# Autodesk Inventor assembly: Main Body
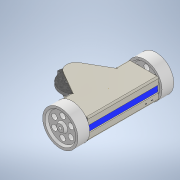
[picture p0: Inventor's stored thumbnail of the model, 180x180]
Saved by Autodesk Inventor 2022 (Build 260153000, 153)
## iProperties
Created: 2022-08-09
Part Number: Main Body
Document SubType Name: Assembly
Designer: Nick
Mass: 1318.27 g
Surface Area: 1845.37 cm^2
Volume: 451.196 cm^3
Density: 2.92172 g/cm^3
Author: Nick
## Documents named in this file (15)
- Y:\Projects\BattleBot\Main Body.iam
- Y:\Projects\BattleBot\Battery.ipt
- Y:\Projects\BattleBot\ESC.ipt
- Y:\Projects\BattleBot\Motor.ipt
- Y:\Projects\BattleBot\RC Reciever.ipt
- Y:\Projects\BattleBot\Base Plate.ipt
- Y:\Projects\BattleBot\Weapon.ipt
- Y:\Projects\BattleBot\Unmodified Motor.ipt
- Y:\Projects\BattleBot\Brushed ESC.ipt
- Y:\Projects\BattleBot\Motor Mount.ipt
- Y:\Projects\BattleBot\Wheel.ipt
- Y:\Projects\BattleBot\6201 Bearing.ipt
- Y:\Projects\BattleBot\Pulley.ipt
- Y:\Projects\BattleBot\6901 Bearing.ipt
- Y:\Projects\BattleBot\pulley flange.ipt
## Components (19 placed, 14 different names)
1. Battery:1 — Mate:65, Mate:66
2. ESC:1 — Mate:66
3. RC Reciever:1 — Mate:53, Mate:62, Mate:64
4. Base Plate:1 — Flush:16, Mate:42, Mate:67, Insert:10
5. Weapon:1 — Insert:3, Mate:70
6. Unmodified Motor:1 — Mate:61
7. Motor:2 — Mate:65, Insert:5, Insert:8
8. Motor:3 — Insert:2, Insert:4
9. Brushed ESC:1
10. Brushed ESC:2 — Mate:55, Mate:56, Mate:63
11. Motor Mount:2 — Insert:2, Flush:16, Mate:42, Mate:53, Mate:55, Mate:56, Mate:62, Mate:63, Mate:64, Mate:67, Insert:8, Mate:68, Mate:69, Flush:17
12. Base Plate:2 — Mate:61, Insert:3, Insert:7, Mate:68, Mate:69, Flush:17
13. Wheel:1 — Insert:5
14. Wheel:2 — Insert:4
15. 6201 Bearing:2 — Insert:7
16. Pulley:1 — Insert:11, Mate:70, Insert:13, Insert:14
17. 6901 Bearing:1 — Insert:10, Insert:14
18. pulley flange:1 — Insert:11
19. pulley flange:2 — Insert:13
## Relationships (26: Mate 14, Insert 10, Flush 2)
- Insert:2: Motor:3 ↔ Motor Mount:2
- Flush:16: Base Plate:1 ↔ Motor Mount:2
- Mate:42: Base Plate:1 ↔ Motor Mount:2
- Mate:53: RC Reciever:1 ↔ Motor Mount:2
- Mate:55: Brushed ESC:2 ↔ Motor Mount:2
- Mate:56: Brushed ESC:2 ↔ Motor Mount:2
- Mate:61: Unmodified Motor:1 ↔ Base Plate:2
- Insert:3 (16.825 mm): Weapon:1 ↔ Base Plate:2
- Mate:62: RC Reciever:1 ↔ Motor Mount:2
- Mate:63 (5 mm): Brushed ESC:2 ↔ Motor Mount:2
- Mate:64: RC Reciever:1 ↔ Motor Mount:2
- Mate:65 (6 mm): Battery:1 ↔ Motor:2
- Mate:66 (3 mm): Battery:1 ↔ ESC:1
- Mate:67: Base Plate:1 ↔ Motor Mount:2
- Insert:4 (2 mm): Motor:3 ↔ Wheel:2
- Insert:5 (2 mm): Motor:2 ↔ Wheel:1
- Insert:7: Base Plate:2 ↔ 6201 Bearing:2
- Insert:8: Motor:2 ↔ Motor Mount:2
- Mate:68: Motor Mount:2 ↔ Base Plate:2
- Mate:69: Motor Mount:2 ↔ Base Plate:2
- Flush:17: Motor Mount:2 ↔ Base Plate:2
- Insert:10: Base Plate:1 ↔ 6901 Bearing:1
- Insert:11: Pulley:1 ↔ pulley flange:1
- Mate:70: Weapon:1 ↔ Pulley:1
- Insert:13: Pulley:1 ↔ pulley flange:2
- Insert:14: Pulley:1 ↔ 6901 Bearing:1
